# Autodesk Inventor assembly: Servo block + gear
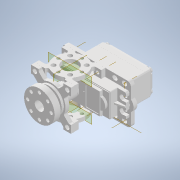
[picture p0: Inventor's stored thumbnail of the model, 180x180]
Saved by Autodesk Inventor 2020 (Build 240168000, 168)
## iProperties
Created: 2020-01-01
Part Number: Servo block + gear
Document SubType Name: Assembly
Designer: ball
Author: ball
## Documents named in this file (3)
- D:\FTC8863\2019 Robot\Collection\Servo block + gear.iam
- D:\FTC8863\Actobotics\637 parts\637112 servo block 25 spline.iam
- D:\FTC8863\Actobotics\615 parts\615190.ipt
## Components (2 placed, 2 different names)
1. 637112 servo block 25 spline:1 [sub-assembly] — Mate:1, Mate:2, Mate:3
2. 615190:1 — Mate:1, Mate:2, Mate:3
## Relationships (3: Mate 3)
- Mate:1: 637112 servo block 25 spline:1 ↔ 615190:1
- Mate:2: 637112 servo block 25 spline:1 ↔ 615190:1
- Mate:3: 637112 servo block 25 spline:1 ↔ 615190:1
